# Autodesk Inventor assembly: assembly_holder3
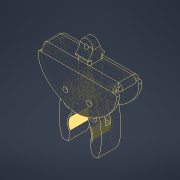
[picture p0: Inventor's stored thumbnail of the model, 180x180]
Saved by Autodesk Inventor 2021 (Build 250183000, 183)
## iProperties
Created: 2021-06-13
Part Number: assembly_holder3
Document SubType Name: Assembly
Designer: Watchdog
Mass: 463.136 g
Surface Area: 313.479 cm^2
Volume: 58.76 cm^3
Density: 7.88182 g/cm^3
Author: Watchdog
## Documents named in this file (13)
- C:\Users\Watchdog\OneDrive - Flinders\Advn Mech Design Shared\6_Development\2_Design\inventor\securing_mechanism\securingMechanism_variant_vertical_x\assembly_holder3.iam
- C:\Users\Watchdog\OneDrive - Flinders\Advn Mech Design Shared\6_Development\2_Design\inventor\securing_mechanism\securingMechanism_variant_vertical_x\holder3_l2.ipt
- C:\Users\Watchdog\OneDrive - Flinders\Advn Mech Design Shared\6_Development\2_Design\inventor\securing_mechanism\securingMechanism_variant_vertical_x\holder3_l3.ipt
- C:\Users\Watchdog\OneDrive - Flinders\Advn Mech Design Shared\6_Development\2_Design\inventor\securing_mechanism\securingMechanism_variant_vertical_x\holder3_l4.ipt
- C:\Users\Watchdog\OneDrive - Flinders\Advn Mech Design Shared\6_Development\2_Design\inventor\securing_mechanism\securingMechanism_variant_vertical_x\holder3_l1_sheetmetal.ipt
- C:\Users\Watchdog\OneDrive - Flinders\Advn Mech Design Shared\6_Development\2_Design\inventor\securing_mechanism\securingMechanism_variant_vertical_x\testCylinder.ipt
- C:\Users\Watchdog\OneDrive - Flinders\Advn Mech Design Shared\6_Development\2_Design\inventor\securing_mechanism\securingMechanism_variant_vertical_x\holder3_cushion.ipt
- C:\Users\Watchdog\OneDrive - Flinders\Advn Mech Design Shared\6_Development\2_Design\inventor\securing_mechanism\securingMechanism_variant_vertical_x\assembly_holder3\AIP\FEA\dmwzxlnts.fins
- C:\Users\Watchdog\OneDrive - Flinders\Advn Mech Design Shared\6_Development\2_Design\inventor\securing_mechanism\securingMechanism_variant_vertical_x\assembly_holder3\AIP\FEA\dmwzxlnts.fsat
- C:\Users\Watchdog\OneDrive - Flinders\Advn Mech Design Shared\6_Development\2_Design\inventor\securing_mechanism\securingMechanism_variant_vertical_x\assembly_holder3\AIP\FEA\dmwzxlnts.ftes
- C:\Users\Watchdog\OneDrive - Flinders\Advn Mech Design Shared\6_Development\2_Design\inventor\securing_mechanism\securingMechanism_variant_vertical_x\assembly_holder3\AIP\FEA\dmwzxlnts.fwiz
- C:\Users\Watchdog\OneDrive - Flinders\Advn Mech Design Shared\6_Development\2_Design\inventor\securing_mechanism\securingMechanism_variant_vertical_x\assembly_holder3\AIP\FEA\dmwzxlny8.fmsh
- C:\Users\Watchdog\OneDrive - Flinders\Advn Mech Design Shared\6_Development\2_Design\inventor\securing_mechanism\securingMechanism_variant_vertical_x\assembly_holder3\AIP\FEA\dmwzxlny9.fres
## Components (9 placed, 6 different names)
1. holder3_l4:1 — Cylindrical:1, Mate:7, Mate:16, Mate:17
2. holder3_l3:1 — Cylindrical:1, Mate:7, Rotational:1, Cylindrical:2, Mate:12
3. holder3_l3:2 — Rotational:1, Cylindrical:3, Mate:14
4. holder3_l2:1 — Cylindrical:2, Mate:12, Cylindrical:4, Flush:3, Mate:19, Flush:4, Mate:21
5. holder3_l2:2 — Cylindrical:3, Mate:14, Cylindrical:5, Mate:20, Flush:5, Mate:22
6. holder3_l1_sheetmetal:1 — Mate:15, Flush:1, Flush:2, Mate:16, Mate:17, Cylindrical:4, Cylindrical:5
7. testCylinder:1 — Flush:3, Mate:18
8. holder3_cushion:1 — Mate:19, Flush:4, Mate:21
9. holder3_cushion:2 — Mate:20, Flush:5, Mate:22
## Relationships (22: Mate 11, CylindricalJoint 5, Flush 5, RevoluteJoint 1)
- Cylindrical:1: holder3_l4:1 ↔ holder3_l3:1
- Mate:7: holder3_l4:1 ↔ holder3_l3:1
- Rotational:1 [RevoluteJoint]: holder3_l3:1 ↔ holder3_l3:2
- Cylindrical:2: holder3_l3:1 ↔ holder3_l2:1
- Cylindrical:3: holder3_l3:2 ↔ holder3_l2:2
- Mate:12: holder3_l3:1 ↔ holder3_l2:1
- Mate:14: holder3_l3:2 ↔ holder3_l2:2
- Mate:15: holder3_l1_sheetmetal:1
- Flush:1: holder3_l1_sheetmetal:1
- Flush:2: holder3_l1_sheetmetal:1
- Mate:16: holder3_l4:1 ↔ holder3_l1_sheetmetal:1
- Mate:17: holder3_l4:1 ↔ holder3_l1_sheetmetal:1
- Cylindrical:4: holder3_l2:1 ↔ holder3_l1_sheetmetal:1
- Cylindrical:5: holder3_l2:2 ↔ holder3_l1_sheetmetal:1
- Flush:3: holder3_l2:1 ↔ testCylinder:1
- Mate:18: testCylinder:1
- Mate:19: holder3_l2:1 ↔ holder3_cushion:1
- Mate:20: holder3_l2:2 ↔ holder3_cushion:2
- Flush:4: holder3_l2:1 ↔ holder3_cushion:1
- Flush:5: holder3_l2:2 ↔ holder3_cushion:2
- Mate:21: holder3_l2:1 ↔ holder3_cushion:1
- Mate:22: holder3_l2:2 ↔ holder3_cushion:2
## Named parameters: sa_0 = 0, sa_1 = -9810, sa_2 = 0
note: some values were not read from the file. Shown as the stored number, unit unknown: "sa_0", "sa_1", "sa_2".
